# Autodesk Inventor assembly: Assembly9
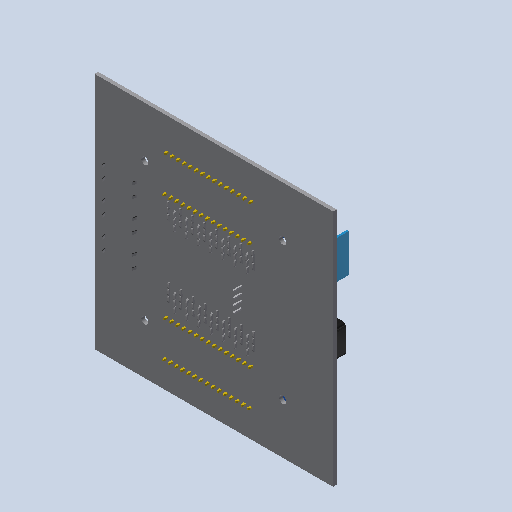
[picture p0: Inventor's stored thumbnail of the model, 512x512]
Saved by Autodesk Inventor 2024 (Build 280153000, 153)
## iProperties
Created: 2023-04-17
Part Number: Assembly9
Document SubType Name: Assembly
Designer: Analuam
Author: Analuam
## Documents named in this file (12)
- D:\Dek Diyah\Assembly9.iam
- D:\Dek Diyah\PCB_sheald.ipt
- F:\Inventor part\Tactal Switch - THRU(12mmx12mmx8mm)-Black.ipt
- F:\Inventor part\Tactal Switch - THRU(12mmx12mmx8mm)-Blue.ipt
- F:\Inventor part\Tactal Switch - THRU(12mmx12mmx8mm)-Brown.ipt
- F:\Inventor part\Pin Header\15er Pin Header Female.ipt
- F:\Inventor part\Arduino\Arduino Nano.iam
- F:\Inventor part\lm2596.ipt
- F:\Inventor part\HMC5883L\HMC5883L.iam
- F:\Inventor part\MCP9808.iam
- F:\Inventor part\Header - SMD - Vertical - 15.ipt
- F:\Inventor part\Capteur bleutooth\Capteur Blautooth.iam
## Components (20 placed, 11 different names)
1. PCB_sheald:1 — Mate:1, Flush:1, Flush:2, Mate:2, Flush:3, Flush:4, Mate:3, Flush:5, Flush:6, Mate:6, Mate:9, Mate:10, Mate:11, Mate:12, Mate:13, Mate:14, Mate:15, Mate:16, Mate:17, Mate:18, Mate:19, Flush:17
2. Tactal Switch - THRU(12mmx12mmx8mm)-Black:1 — Mate:3, Flush:5, Flush:6
3. Tactal Switch - THRU(12mmx12mmx8mm)-Blue:1 — Mate:2, Flush:3, Flush:4
4. Tactal Switch - THRU(12mmx12mmx8mm)-Brown:1 — Mate:1, Flush:1, Flush:2
5. 15er Pin Header Female:1 — Flush:7, Flush:8, Flush:9, Mate:4, Mate:6
6. 15er Pin Header Female:2 — Flush:10, Flush:11, Mate:5
7. Arduino Nano:2 [sub-assembly] — Flush:7, Flush:8, Flush:9, Mate:4, Flush:10, Flush:11, Mate:5
8. 15er Pin Header Female:3 — Mate:9
9. 15er Pin Header Female:4
10. Arduino Nano:3 [sub-assembly]
11. lm2596:1 — Mate:10
12. HMC5883L:1 [sub-assembly] — Mate:11
13. MCP9808:2 [sub-assembly] — Mate:12
14. Header - SMD - Vertical - 15:1 — Mate:13
15. Header - SMD - Vertical - 15:2 — Mate:14
16. Header - SMD - Vertical - 15:3 — Mate:15
17. Header - SMD - Vertical - 15:4 — Mate:18
18. Header - SMD - Vertical - 15:5 — Mate:17
19. Header - SMD - Vertical - 15:6 — Mate:16
20. Capteur Blautooth:1 [sub-assembly] — Mate:19, Flush:17
## Relationships (36: Mate 19, Flush 17)
- Mate:1: PCB_sheald:1 ↔ Tactal Switch - THRU(12mmx12mmx8mm)-Brown:1
- Flush:1 (40 mm): PCB_sheald:1 ↔ Tactal Switch - THRU(12mmx12mmx8mm)-Brown:1
- Flush:2 (5 mm): PCB_sheald:1 ↔ Tactal Switch - THRU(12mmx12mmx8mm)-Brown:1
- Mate:2: PCB_sheald:1 ↔ Tactal Switch - THRU(12mmx12mmx8mm)-Blue:1
- Flush:3 (5 mm): PCB_sheald:1 ↔ Tactal Switch - THRU(12mmx12mmx8mm)-Blue:1
- Flush:4 (27 mm): PCB_sheald:1 ↔ Tactal Switch - THRU(12mmx12mmx8mm)-Blue:1
- Mate:3: PCB_sheald:1 ↔ Tactal Switch - THRU(12mmx12mmx8mm)-Black:1
- Flush:5 (5 mm): PCB_sheald:1 ↔ Tactal Switch - THRU(12mmx12mmx8mm)-Black:1
- Flush:6 (53 mm): PCB_sheald:1 ↔ Tactal Switch - THRU(12mmx12mmx8mm)-Black:1
- Flush:7: 15er Pin Header Female:1 ↔ Arduino Nano:2
- Flush:8: 15er Pin Header Female:1 ↔ Arduino Nano:2
- Flush:9: 15er Pin Header Female:1 ↔ Arduino Nano:2
- Mate:4: 15er Pin Header Female:1 ↔ Arduino Nano:2
- Flush:10: 15er Pin Header Female:2 ↔ Arduino Nano:2
- Flush:11: 15er Pin Header Female:2 ↔ Arduino Nano:2
- Mate:5: 15er Pin Header Female:2 ↔ Arduino Nano:2
- Mate:6: PCB_sheald:1 ↔ 15er Pin Header Female:1
- [Flush]: 15er Pin Header Female:3 ↔ Arduino Nano:3
- [Flush]: 15er Pin Header Female:3 ↔ Arduino Nano:3
- [Flush]: 15er Pin Header Female:3 ↔ Arduino Nano:3
- [Mate]: 15er Pin Header Female:3 ↔ Arduino Nano:3
- [Flush]: 15er Pin Header Female:4 ↔ Arduino Nano:3
- [Flush]: 15er Pin Header Female:4 ↔ Arduino Nano:3
- [Mate]: 15er Pin Header Female:4 ↔ Arduino Nano:3
- Mate:9: PCB_sheald:1 ↔ 15er Pin Header Female:3
- Mate:10: PCB_sheald:1 ↔ lm2596:1
- Mate:11: PCB_sheald:1 ↔ HMC5883L:1
- Mate:12: PCB_sheald:1 ↔ MCP9808:2
- Mate:13: PCB_sheald:1 ↔ Header - SMD - Vertical - 15:1
- Mate:14: PCB_sheald:1 ↔ Header - SMD - Vertical - 15:2
- Mate:15: PCB_sheald:1 ↔ Header - SMD - Vertical - 15:3
- Mate:16: PCB_sheald:1 ↔ Header - SMD - Vertical - 15:6
- Mate:17: PCB_sheald:1 ↔ Header - SMD - Vertical - 15:5
- Mate:18: PCB_sheald:1 ↔ Header - SMD - Vertical - 15:4
- Mate:19: PCB_sheald:1 ↔ Capteur Blautooth:1
- Flush:17 (32 mm): PCB_sheald:1 ↔ Capteur Blautooth:1
## Named parameters: d27_d15 = 0 mm, d28_d16 = 0 mm, d29_d17 = 0 mm, d30_d18 = 0 mm, d31_d12 = 0 mm, d32_d13 = 0 mm, d33_d14 = 0 mm
